# Autodesk Inventor assembly: Sistema movimiento derecho
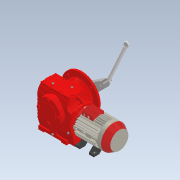
[picture p0: Inventor's stored thumbnail of the model, 180x180]
Saved by Autodesk Inventor 2021 (Build 250183000, 183)
## iProperties
Created: 2021-06-19
Part Number: Sistema movimiento derecho
Document SubType Name: Assembly
Designer: Andrés Holguín
Author: Andrés Holguín
## Documents named in this file (7)
- C:\Users\andre\Documents\GitHub\Dis.-Mecatronico-E6\inventor proyecto\Motores y reductores\Sistema movimiento derecho.iam
- C:\Users\andre\Documents\GitHub\Dis.-Mecatronico-E6\inventor proyecto\Motores y reductores\Reductor Derecha.iam
- Reductor Derecha.iam
- C:\Users\andre\Documents\GitHub\Dis.-Mecatronico-E6\inventor proyecto\Motores y reductores\pasador.ipt
- C:\Users\andre\Documents\GitHub\Dis.-Mecatronico-E6\inventor proyecto\Motores y reductores\Biela Completa.iam
- C:\Users\andre\Documents\GitHub\Dis.-Mecatronico-E6\inventor proyecto\Motores y reductores\placa manivela.ipt
- C:\Users\andre\Documents\GitHub\Dis.-Mecatronico-E6\inventor proyecto\Motores y reductores\Motor Simens Frame 112M IM B3.ipt
## Components (5 placed, 5 different names)
1. Reductor Derecha:1 [sub-assembly] — Insert:1, Mate:1, Rigid:1
2. pasador:1 — Insert:2, Insert:3
3. Biela Completa:1 [sub-assembly] — Insert:3
4. placa manivela:1 — Insert:1, Mate:1, Insert:2
5. Motor Simens Frame 112M IM B3:1 — Rigid:1
## Relationships (5: Insert 3, Mate 1, WeldJoint 1)
- Insert:1 (50 mm): Reductor Derecha:1 ↔ placa manivela:1
- Mate:1: Reductor Derecha:1 ↔ placa manivela:1
- Insert:2: pasador:1 ↔ placa manivela:1
- Insert:3 (15 mm): pasador:1 ↔ Biela Completa:1
- Rigid:1 [WeldJoint]: Reductor Derecha:1 ↔ Motor Simens Frame 112M IM B3:1
